# Autodesk Inventor assembly: Assembly1
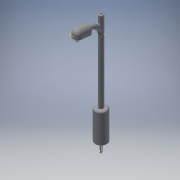
[picture p0: Inventor's stored thumbnail of the model, 180x180]
Saved by Autodesk Inventor 2018 (Build 220112000, 112)
## iProperties
Created: 2018-12-13
Part Number: Assembly1
Document SubType Name: Assembly
Designer: petal
Author: petal
## Documents named in this file (6)
- D:\OneDrive\Dokumenty\Assembly1.iam
- D:\OneDrive\Dokumenty\lampa.ipt
- D:\OneDrive\Dokumenty\3,5mm jack.ipt
- D:\OneDrive\3D modely\Grasshopper\Grasshopper\ledka.ipt
- D:\OneDrive\Dokumenty\lampa_MIR.ipt
- D:\OneDrive\3D modely\Grasshopper\Grasshopper\Part4.ipt
## Components (5 placed, 5 different names)
1. lampa:1 — Mate:1, Mate:2, Mate:3, Flush:1
2. 3,5mm jack:1 — Mate:1
3. ledka:1 — Mate:2, Mate:3
4. lampa_MIR:1
5. Part4:1 — Flush:1
## Relationships (4: Mate 3, Flush 1)
- Mate:1: lampa:1 ↔ 3,5mm jack:1
- Mate:2: lampa:1 ↔ ledka:1
- Mate:3: lampa:1 ↔ ledka:1
- Flush:1: lampa:1 ↔ Part4:1
